# Autodesk Inventor assembly: Main_assy
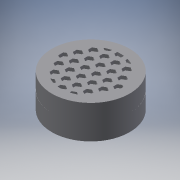
[picture p0: Inventor's stored thumbnail of the model, 180x180]
Saved by Autodesk Inventor 2017 (Build 210142000, 142)
## iProperties
Created: 2019-05-26
Part Number: Main_assy
Document SubType Name: Assembly
Designer: Mitch
Author: Mitch
## Documents named in this file (6)
- E:\Youtube Channel\Pojects\Scammer Away\Mech\Main_assy.iam
- E:\Youtube Channel\Pojects\Scammer Away\Mech\Bottom.ipt
- E:\Youtube Channel\Pojects\Scammer Away\Mech\electronics_assy.iam
- E:\Youtube Channel\Pojects\Scammer Away\Mech\top.ipt
- E:\Youtube Channel\Pojects\Scammer Away\Mech\tactileswitch-short.ipt
- E:\Youtube Channel\Pojects\Scammer Away\Mech\Button.ipt
## Components (5 placed, 5 different names)
1. Bottom:1 — Mate:1, Mate:2, Mate:3, Mate:4, Mate:5, Tangent:1, Tangent:2
2. electronics_assy:1 [sub-assembly] — Mate:1, Mate:2
3. top:1 — Mate:3, Mate:4
4. tactileswitch-short:1 — Mate:5, Tangent:1, Tangent:2, Mate:6
5. Button:1 — Mate:6
## Relationships (8: Mate 6, Tangent 2)
- Mate:1: Bottom:1 ↔ electronics_assy:1
- Mate:2 (0.4318 mm): Bottom:1 ↔ electronics_assy:1
- Mate:3: Bottom:1 ↔ top:1
- Mate:4: Bottom:1 ↔ top:1
- Mate:5: Bottom:1 ↔ tactileswitch-short:1
- Tangent:1 (-22.6949 mm): Bottom:1 ↔ tactileswitch-short:1
- Tangent:2 (-34.925 mm): Bottom:1 ↔ tactileswitch-short:1
- Mate:6: tactileswitch-short:1 ↔ Button:1
